# Autodesk Inventor assembly: D2MG
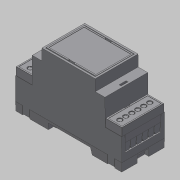
[picture p0: Inventor's stored thumbnail of the model, 180x180]
Saved by Autodesk Inventor 2018 (Build 220112000, 112)
## iProperties
Created: 2015-02-09
Part Number: D2MG
Document SubType Name: Assembly
Designer: Abbath
Author: Abbath
## Documents named in this file (5)
- D:\Abbath\03 RaceIt WorkSpace\Библиотеки\!3D модели\Корпуса приборные\Gainta\D2MG\3D\Inv\D2MG.iam
- D:\Abbath\03 RaceIt WorkSpace\Библиотеки\!3D модели\Корпуса приборные\Gainta\D2MG\3D\Inv\D2MG-BODY.ipt
- D:\Abbath\03 RaceIt WorkSpace\Библиотеки\!3D модели\Корпуса приборные\Gainta\D2MG\3D\Inv\D2MG-BASE.ipt
- D:\Abbath\03 RaceIt WorkSpace\Библиотеки\!3D модели\Корпуса приборные\Gainta\D2MG\3D\Inv\D2MG-GUARD.ipt
- D:\Abbath\03 RaceIt WorkSpace\Библиотеки\!3D модели\Корпуса приборные\Gainta\D2MG\3D\Inv\D2MG-COVER.ipt
## Components (5 placed, 4 different names)
1. D2MG-BASE:1 — Заподлицо:1, Заподлицо:2, Совмещение:1, Совмещение:2, Заподлицо:3
2. D2MG-BODY:1 — Заподлицо:1, Заподлицо:2, Совмещение:1, Совмещение:3, Совмещение:4, Совмещение:5, Совмещение:6, Совмещение:7, Заподлицо:4, Совмещение:8
3. D2MG-GUARD:1 — Совмещение:2, Совмещение:3, Совмещение:4
4. D2MG-GUARD:2 — Заподлицо:3, Совмещение:5, Совмещение:6
5. D2MG-COVER:1 — Совмещение:7, Заподлицо:4, Совмещение:8
## Relationships (12: Mate 8, Flush 4)
- Заподлицо:1 [Flush]: D2MG-BASE:1 ↔ D2MG-BODY:1
- Заподлицо:2 [Flush]: D2MG-BASE:1 ↔ D2MG-BODY:1
- Совмещение:1 [Mate]: D2MG-BASE:1 ↔ D2MG-BODY:1
- Совмещение:2 [Mate]: D2MG-BASE:1 ↔ D2MG-GUARD:1
- Совмещение:3 [Mate]: D2MG-BODY:1 ↔ D2MG-GUARD:1
- Совмещение:4 [Mate]: D2MG-BODY:1 ↔ D2MG-GUARD:1
- Заподлицо:3 [Flush]: D2MG-BASE:1 ↔ D2MG-GUARD:2
- Совмещение:5 [Mate]: D2MG-BODY:1 ↔ D2MG-GUARD:2
- Совмещение:6 [Mate]: D2MG-BODY:1 ↔ D2MG-GUARD:2
- Совмещение:7 [Mate]: D2MG-BODY:1 ↔ D2MG-COVER:1
- Заподлицо:4 [Flush]: D2MG-BODY:1 ↔ D2MG-COVER:1
- Совмещение:8 [Mate]: D2MG-BODY:1 ↔ D2MG-COVER:1
